# Autodesk Inventor assembly: belt_print
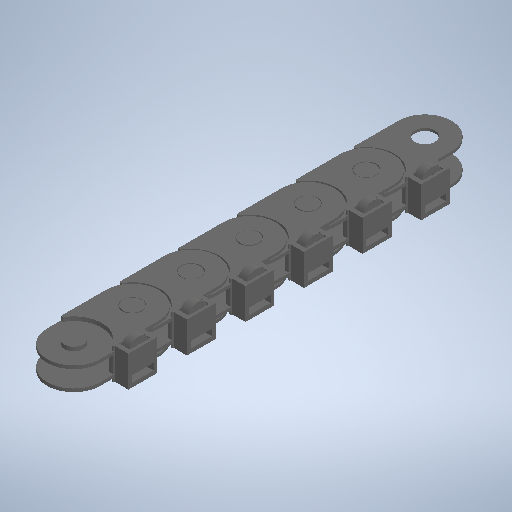
[picture p0: Inventor's stored thumbnail of the model, 512x512]
Saved by Autodesk Inventor 2026.1 (Build 301233020, 233B)
## iProperties
Created: 2025-09-27
Part Number: belt_print
Document SubType Name: Assembly
Designer: hibik
Author: hibik
## Documents named in this file (2)
- C:\Users\hibik\Documents\Robomech\conveyer\belt\belt_print.iam
- C:\Users\hibik\Documents\Robomech\conveyer\belt\belt.ipt
## Components (6 placed, 1 different names)
1. belt:1 — 挿入:1, 角度:9, 挿入:21, フラッシュ:1
2. belt:2 — 挿入:1, 挿入:2, 角度:9, 角度:10
3. belt:3 — 挿入:2, 角度:10
4. belt:10
5. belt:11
6. belt:12 — 挿入:21, フラッシュ:1
## Relationships (10: Insert 5, Angle 4, Flush 1)
- 挿入:1 [Insert] (0.6 mm): belt:1 ↔ belt:2
- 挿入:2 [Insert] (0.6 mm): belt:2 ↔ belt:3
- 角度:9 [Angle] (0 deg): belt:1 ↔ belt:2
- 角度:10 [Angle] (0 deg): belt:2 ↔ belt:3
- [Insert] (0.6 mm): belt:10 ↔ belt:11
- [Insert] (0.6 mm): belt:11 ↔ belt:12
- [Angle] (0 deg): belt:10 ↔ belt:11
- [Angle] (0 deg): belt:11 ↔ belt:12
- 挿入:21 [Insert] (-0.6 mm): belt:1 ↔ belt:12
- フラッシュ:1 [Flush]: belt:1 ↔ belt:12
## Named parameters: d62_d0 = 0.6 mm, d63_d1 = 0.6 mm, d64_d24 = 0 deg, d65_d25 = 0 deg
